# Autodesk Inventor assembly: Track v3 Assy
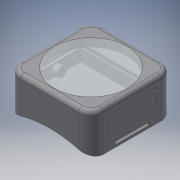
[picture p0: Inventor's stored thumbnail of the model, 180x180]
Saved by Autodesk Inventor 2016 (Build 200138000, 138)
## iProperties
Created: 2016-05-24
Part Number: Track v3 Assy
Document SubType Name: Assembly
Designer: xdlea
Author: xdlea
## Documents named in this file (5)
- D:\Library\Documents\4-3D Models\Track v3 Assy.iam
- D:\Library\Documents\4-3D Models\Track v3 Button.ipt
- D:\Library\Documents\4-3D Models\Track v3.ipt
- D:\Library\Documents\4-3D Models\Track v3 Cover.ipt
- D:\Library\Documents\4-3D Models\Track v3 Access Cover.ipt
## Components (4 placed, 4 different names)
1. Track v3 Button:1 — Mate:1, Mate:2
2. Track v3:1 — Mate:1, Mate:2, Mate:3, Mate:4, Mate:5, Flush:1, Mate:6
3. Track v3 Cover:1 — Mate:3, Mate:4
4. Track v3 Access Cover:1 — Mate:5, Flush:1, Mate:6
## Relationships (7: Mate 6, Flush 1)
- Mate:1: Track v3 Button:1 ↔ Track v3:1
- Mate:2: Track v3 Button:1 ↔ Track v3:1
- Mate:3: Track v3:1 ↔ Track v3 Cover:1
- Mate:4: Track v3:1 ↔ Track v3 Cover:1
- Mate:5: Track v3:1 ↔ Track v3 Access Cover:1
- Flush:1: Track v3:1 ↔ Track v3 Access Cover:1
- Mate:6: Track v3:1 ↔ Track v3 Access Cover:1
